# Autodesk Inventor assembly: PrintedPully2Halves
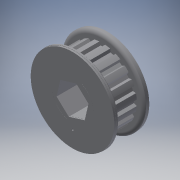
[picture p0: Inventor's stored thumbnail of the model, 180x180]
Saved by Autodesk Inventor 2019 (Build 230136000, 136)
## iProperties
Created: 2019-02-15
Part Number: PrintedPully2Halves
Document SubType Name: Assembly
Designer: james
Author: james
## Documents named in this file (3)
- F:\JimsDesign\2019CHS4089\PrintedPully2Halves.iam
- F:\JimsDesign\2019CHS4089\PullyHex.ipt
- F:\JimsDesign\2019CHS4089\PullyShell2Part.ipt
## Components (4 placed, 2 different names)
1. PullyShell2Part:1 — Mate:1, Mate:2, Mate:3, Mate:5, Flush:2
2. PullyShell2Part:2 — Mate:1, Mate:2, Mate:3, Flush:4
3. PullyHex:1 — Mate:4, Flush:2, Flush:5
4. PullyHex:2 — Mate:4, Mate:5, Flush:4, Flush:5
## Relationships (8: Mate 5, Flush 3)
- Mate:1: PullyShell2Part:1 ↔ PullyShell2Part:2
- Mate:2: PullyShell2Part:1 ↔ PullyShell2Part:2
- Mate:3 (-15.875 mm): PullyShell2Part:1 ↔ PullyShell2Part:2
- Mate:4: PullyHex:1 ↔ PullyHex:2
- Mate:5: PullyShell2Part:1 ↔ PullyHex:2
- Flush:2: PullyShell2Part:1 ↔ PullyHex:1
- Flush:4: PullyShell2Part:2 ↔ PullyHex:2
- Flush:5: PullyHex:1 ↔ PullyHex:2
